# Autodesk Inventor assembly: 3.25" Traction Wheel, Square Insert
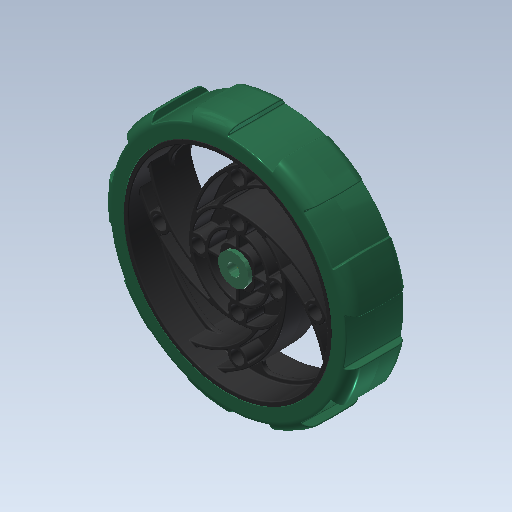
[picture p0: Inventor's stored thumbnail of the model, 512x512]
Saved by Autodesk Inventor 2020 (Build 240168000, 168)
## iProperties
Created: 2014-08-29
Document SubType Name: Assembly
Designer: Jordan Kiesel
Vendor: VEX Robotics, Inc.
Mass: 54.4672 g
Surface Area: 417.393 cm^2
Volume: 47.139 cm^3
Density: 1.15546 g/cm^3
Company: Bots 'n' Stuff
Author: Jordan Kiesel
Title: 3.25" Traction Wheel, Square Insert
## Documents named in this file (3)
- D:\Robotics\CAD\2018 BNS-VRC-SID Library\Motion\Wheels _ Rollers\3.25_ Traction Wheel, Free Spinning Insert.iam
- D:\Robotics\CAD\2018 BNS-VRC-SID Library\Motion\Wheels _ Rollers\Reference Parts\3.25_ Traction Wheels\3.25_ Traction Wheel.iam
- D:\Robotics\CAD\2018 BNS-VRC-SID Library\Motion\Reference Parts\Free Spinning Gear Insert.ipt
## Components (3 placed, 2 different names)
1. 3.25_ Traction Wheel:1 [sub-assembly] — Mate:3, Mate:6
2. Free Spinning Gear Insert:1 — Mate:3
3. Free Spinning Gear Insert:2 — Mate:6
## Relationships (6: Mate 6)
- [Mate] (0.0254 mm): 3.25_ Traction Wheel:1 ↔ Free Spinning Gear Insert:1
- [Mate] (0.0254 mm): 3.25_ Traction Wheel:1 ↔ Free Spinning Gear Insert:1
- Mate:3: 3.25_ Traction Wheel:1 ↔ Free Spinning Gear Insert:1
- [Mate] (0.0254 mm): 3.25_ Traction Wheel:1 ↔ Free Spinning Gear Insert:2
- [Mate] (0.0254 mm): 3.25_ Traction Wheel:1 ↔ Free Spinning Gear Insert:2
- Mate:6: 3.25_ Traction Wheel:1 ↔ Free Spinning Gear Insert:2
